# Autodesk Inventor assembly: MG-958 servo
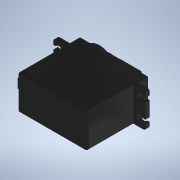
[picture p0: Inventor's stored thumbnail of the model, 180x180]
Saved by Autodesk Inventor 2020 (Build 240168000, 168)
## iProperties
Created: 2021-01-02
Part Number: MG-958 servo
Document SubType Name: Assembly
Designer: Vikki
Title: C:/Users/nithi/OneDrive/Desktop/Fusion 360/996R.step
Sending System: Autodesk Translation Framework v9.7.1.1290
Preprocessor: ST-DEVELOPER v18.1
## Documents named in this file (5)
- D:\borewell rescuebot\pll manipulator files\sps manipulator\MG-958 servo.iam
- D:\borewell rescuebot\pll manipulator files\sps manipulator\Golden part.ipt
- D:\borewell rescuebot\pll manipulator files\sps manipulator\Wires.ipt
- D:\borewell rescuebot\pll manipulator files\sps manipulator\Connector.iam
- D:\borewell rescuebot\pll manipulator files\sps manipulator\Part13.ipt
## Components (4 placed, 4 different names)
1. Golden part:1 — Mate:1, Mate:2
2. Wires:1
3. Connector:1 [sub-assembly]
4. Part13 — Mate:1, Mate:2
## Relationships (2: Mate 2)
- Mate:1: Golden part:1 ↔ Part13
- Mate:2: Golden part:1 ↔ Part13
